# Autodesk Inventor assembly: Assembly2
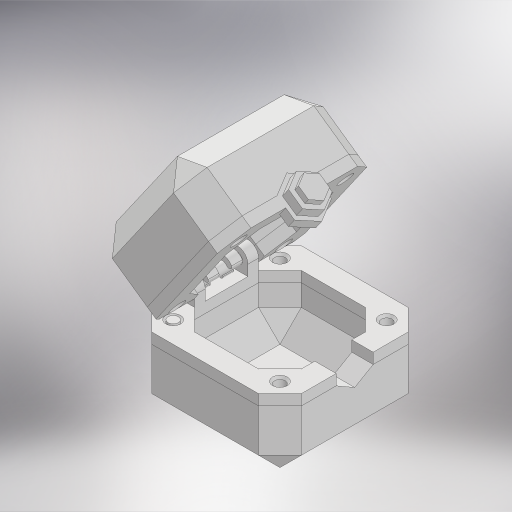
[picture p0: Inventor's stored thumbnail of the model, 512x512]
Saved by Autodesk Inventor 2024 (Build 280153000, 153)
## iProperties
Created: 2023-10-25
Part Number: Assembly2
Document SubType Name: Assembly
Designer: SSAFY
Author: SSAFY
## Documents named in this file (9)
- C:\Users\SSAFY\Desktop\TIL\3D\20231025\Assembly2.iam
- C:\Users\SSAFY\Desktop\TIL\3D\20231025\joint_part_black_2.ipt
- C:\Users\SSAFY\Desktop\TIL\3D\20231025\joint_part_black_8.ipt
- C:\Users\SSAFY\Desktop\TIL\3D\20231025\pokemon_ball_black_part1.ipt
- C:\Users\SSAFY\Desktop\TIL\3D\20231025\pokemon_ball_black_part2.ipt
- C:\Users\SSAFY\Desktop\TIL\3D\20231025\pokemon_ball_red.ipt
- C:\Users\SSAFY\Desktop\TIL\3D\20231025\pokemon_ball_white.ipt
- C:\Users\SSAFY\Desktop\TIL\3D\20231025\white_part1.ipt
- C:\Users\SSAFY\Desktop\TIL\3D\20231025\joint_white_part_1.ipt
## Components (9 placed, 8 different names)
1. joint_part_black_2:1 — Mate:3, Mate:4, Mate:8
2. joint_part_black_2:2 — Mate:6, Mate:7, Mate:9
3. joint_part_black_8:1 — Mate:5, Flush:5
4. pokemon_ball_black_part1:1 — Mate:1, Flush:4, Mate:2, Mate:5, Flush:5, Mate:8, Mate:9
5. pokemon_ball_black_part2:1 — Mate:10, Flush:7, Mate:11, Mate:14, Mate:15
6. pokemon_ball_red:1 — Mate:3, Mate:4, Mate:6, Mate:7, Flush:6, Mate:10, Flush:7, Mate:11
7. pokemon_ball_white:1 — Flush:1, Flush:2, Flush:3, Mate:1, Flush:4, Mate:2, Flush:6
8. white_part1:1 — Mate:12, Mate:13, Mate:14
9. joint_white_part_1:1 — Mate:12, Mate:13, Mate:15
## Relationships (22: Mate 15, Flush 7)
- Flush:1 (9.529 mm): pokemon_ball_white:1
- Flush:2 (-52.514 mm): pokemon_ball_white:1
- Flush:3 (23.95 mm): pokemon_ball_white:1
- Mate:1: pokemon_ball_black_part1:1 ↔ pokemon_ball_white:1
- Flush:4: pokemon_ball_black_part1:1 ↔ pokemon_ball_white:1
- Mate:2: pokemon_ball_black_part1:1 ↔ pokemon_ball_white:1
- Mate:3: joint_part_black_2:1 ↔ pokemon_ball_red:1
- Mate:4 (0.2 mm): joint_part_black_2:1 ↔ pokemon_ball_red:1
- Mate:5: joint_part_black_8:1 ↔ pokemon_ball_black_part1:1
- Flush:5: joint_part_black_8:1 ↔ pokemon_ball_black_part1:1
- Mate:6: joint_part_black_2:2 ↔ pokemon_ball_red:1
- Mate:7 (0.2 mm): joint_part_black_2:2 ↔ pokemon_ball_red:1
- Mate:8: joint_part_black_2:1 ↔ pokemon_ball_black_part1:1
- Mate:9: joint_part_black_2:2 ↔ pokemon_ball_black_part1:1
- Flush:6: pokemon_ball_red:1 ↔ pokemon_ball_white:1
- Mate:10: pokemon_ball_black_part2:1 ↔ pokemon_ball_red:1
- Flush:7: pokemon_ball_black_part2:1 ↔ pokemon_ball_red:1
- Mate:11: pokemon_ball_black_part2:1 ↔ pokemon_ball_red:1
- Mate:12: white_part1:1 ↔ joint_white_part_1:1
- Mate:13: white_part1:1 ↔ joint_white_part_1:1
- Mate:14: pokemon_ball_black_part2:1 ↔ white_part1:1
- Mate:15: pokemon_ball_black_part2:1 ↔ joint_white_part_1:1
